# Autodesk Inventor assembly: Swing_Arm_02
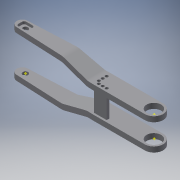
[picture p0: Inventor's stored thumbnail of the model, 180x180]
Saved by Autodesk Inventor 2016 (Build 200138000, 138)
## iProperties
Created: 2016-02-09
Part Number: Swing_Arm_02
Document SubType Name: Assembly
Designer: nils
Author: nils
## Documents named in this file (4)
- D:\bikair\Bikair_CAD-1\Source\Rear_Train\Swing_Arm_02.iam
- D:\bikair\Bikair_CAD-1\Source\Rear_Train\Profile_Straight_MIR_02.ipt
- D:\bikair\Bikair_CAD-1\Source\Rear_Train\Profile_Straight_02.ipt
- D:\bikair\Bikair_CAD-1\Source\Rear_Train\Profile_Middle_02.ipt
## Components (3 placed, 3 different names)
1. Profile_Straight_MIR_02:1 — Mate:1, Mate:2, Mate:3
2. Profile_Straight_02:1 — Mate:1, Mate:2, Mate:3, Mate:4, Mate:5, Mate:6
3. Profile_Middle_02:1 — Mate:4, Mate:5, Mate:6
## Relationships (6: Mate 6)
- Mate:1 (80 mm): Profile_Straight_MIR_02:1 ↔ Profile_Straight_02:1
- Mate:2: Profile_Straight_MIR_02:1 ↔ Profile_Straight_02:1
- Mate:3: Profile_Straight_MIR_02:1 ↔ Profile_Straight_02:1
- Mate:4: Profile_Straight_02:1 ↔ Profile_Middle_02:1
- Mate:5: Profile_Straight_02:1 ↔ Profile_Middle_02:1
- Mate:6: Profile_Straight_02:1 ↔ Profile_Middle_02:1
